# Autodesk Inventor assembly: Assembly
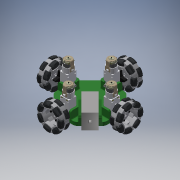
[picture p0: Inventor's stored thumbnail of the model, 180x180]
Saved by Autodesk Inventor 2019 (Build 230136000, 136)
## iProperties
Created: 2018-10-30
Part Number: Assembly
Document SubType Name: Assembly
Designer: Ethan
Author: Ethan
## Documents named in this file (6)
- C:\Users\Ethan\Documents\SE101\3D Models\Assembly.iam
- C:\Users\Ethan\Documents\SE101\3D Models\Motor Solarbotics GM3\Solarbotics-GM3.iam
- C:\Users\Ethan\Documents\SE101\3D Models\Wheel Mount.ipt
- C:\Users\Ethan\Documents\SE101\3D Models\Wheel VEX 228-2536\Wheel VEX 228-2536.iam
- C:\Users\Ethan\Documents\SE101\3D Models\Frame.ipt
- C:\Users\Ethan\Documents\SE101\3D Models\Solenoid.iam
## Components (14 placed, 5 different names)
1. Frame:1 — Flush:1
2. Solenoid:2 [sub-assembly] — Mate:7, Angle:2, Mate:8, Mate:9
3. Solarbotics-GM3:1 [sub-assembly] — Mate:1, Mate:2, Rigid:1
4. Wheel Mount:1 — Rigid:1, Mate:3, Rigid:2
5. Wheel VEX 228-2536:1 [sub-assembly] — Mate:3, Rigid:2
6. Solarbotics-GM3:2 [sub-assembly]
7. Wheel Mount:2
8. Wheel VEX 228-2536:2 [sub-assembly]
9. Solarbotics-GM3:3 [sub-assembly]
10. Wheel Mount:3
11. Wheel VEX 228-2536:3 [sub-assembly]
12. Solarbotics-GM3:4 [sub-assembly]
13. Wheel Mount:4
14. Wheel VEX 228-2536:4 [sub-assembly]
## Component patterns: (4 elements, first: Solarbotics-GM3:1 + Wheel Mount:1 + Wheel VEX 228-2536:1)
## Relationships (10: Mate 6, WeldJoint 2, Flush 1, Angle 1)
- Mate:1 (45 mm): Solarbotics-GM3:1
- Mate:2: Solarbotics-GM3:1
- Rigid:1 [WeldJoint]: Solarbotics-GM3:1 ↔ Wheel Mount:1
- Mate:3: Wheel Mount:1 ↔ Wheel VEX 228-2536:1
- Rigid:2 [WeldJoint] (-2.159 mm): Wheel Mount:1 ↔ Wheel VEX 228-2536:1
- Flush:1: Frame:1
- Mate:7 (-3.135 mm): Solenoid:2
- Angle:2 (45 deg): Solenoid:2
- Mate:8: Solenoid:2
- Mate:9 (-52 mm): Solenoid:2
## Named parameters: motor_outset = 45 mm, solenoid_outset = 52 mm, solenoid_height = -3.135 mm
